# Autodesk Inventor assembly: C-Channel 1x5x1x35 Hole
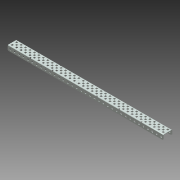
[picture p0: Inventor's stored thumbnail of the model, 180x180]
Saved by Autodesk Inventor 2015 (Build 190159000, 159)
## iProperties
Created: 2017-05-26
Part Number: C-Channel 1x5x1x35 Hole
Document SubType Name: Assembly
Designer: longm
Author: longm
## Documents named in this file (3)
- C:\Users\Tommy\Documents\GitHub\VEX-Robotics-2017-2018\Imperial\Structure\C-Channel 1x5x1x35 Hole.iam
- C:\Users\Tommy\Documents\GitHub\VEX-Robotics-2017-2018\Imperial\Structure\C-Channel 1x2x1x15 Hole.ipt
- C:\Users\Tommy\Documents\GitHub\VEX-Robotics-2017-2018\Imperial\Structure\C-Channel 1x3x1x20 hole.ipt
## Components (2 placed, 2 different names)
1. C-Channel 1x2x1x15 Hole:1 — Mate:1, Flush:1, Flush:2
2. C-Channel 1x3x1x20 hole:1 — Mate:1, Flush:1, Flush:2
## Relationships (3: Flush 2, Mate 1)
- Mate:1: C-Channel 1x2x1x15 Hole:1 ↔ C-Channel 1x3x1x20 hole:1
- Flush:1: C-Channel 1x2x1x15 Hole:1 ↔ C-Channel 1x3x1x20 hole:1
- Flush:2: C-Channel 1x2x1x15 Hole:1 ↔ C-Channel 1x3x1x20 hole:1
